# Autodesk Inventor assembly: servo
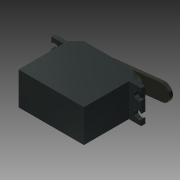
[picture p0: Inventor's stored thumbnail of the model, 180x180]
Saved by Autodesk Inventor 2015 (Build 190159000, 159)
## iProperties
Created: 2015-06-11
Part Number: servo
Document SubType Name: Assembly
Designer: david
Mass: 29.4067 g
Surface Area: 75.1691 cm^2
Volume: 29.4067 cm^3
Density: 1 g/cm^3
Author: david
## Documents named in this file (3)
- Z:\gip\Inventor\generatie 7\motor\servo\servo.iam
- Z:\gip\Inventor\generatie 7\motor\servo\block.ipt
- Z:\gip\Inventor\generatie 7\motor\servo\tang.ipt
## Components (2 placed, 2 different names)
1. block:1 — Mate:1, Mate:2
2. tang:1 — Mate:1, Mate:2
## Relationships (2: Mate 2)
- Mate:1: block:1 ↔ tang:1
- Mate:2: block:1 ↔ tang:1
